# Autodesk Inventor assembly: Outer Tie Rod
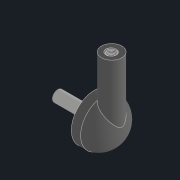
[picture p0: Inventor's stored thumbnail of the model, 180x180]
Saved by Autodesk Inventor 2021 (Build 250183000, 183)
## iProperties
Created: 2020-10-18
Part Number: Outer Tie Rod
Document SubType Name: Assembly
Designer: Eugene Tang
Mass: 63.1047 g
Surface Area: 262.55 cm^2
Volume: 63.1047 cm^3
Density: 1 g/cm^3
Author: Eugene Tang
## Documents named in this file (4)
- C:\Users\teuge\OneDrive - Curtin University of Technology Australia\Y4S2\DFM\Group Project\CAD\Master\Outer Tie Rod.iam
- C:\Users\teuge\OneDrive - Curtin University of Technology Australia\Y4S2\DFM\Group Project\CAD\Master\Outer Tie Rod.ipt
- C:\Users\teuge\OneDrive - Curtin University of Technology Australia\Y4S2\DFM\Group Project\CAD\Parts\Outer Tie Rod Ball.ipt
- C:\Users\teuge\OneDrive - Curtin University of Technology Australia\Y4S2\DFM\Group Project\CAD\Parts\Out Tie Rod Joint Cap.ipt
## Components (3 placed, 3 different names)
1. Outer Tie Rod:1 — Mate:1, Mate:3
2. Outer Tie Rod Ball:1 — Mate:3
3. Out Tie Rod Joint Cap:1 — Mate:1
## Relationships (2: Mate 2)
- Mate:1: Outer Tie Rod:1 ↔ Out Tie Rod Joint Cap:1
- Mate:3: Outer Tie Rod:1 ↔ Outer Tie Rod Ball:1
